# Autodesk Inventor assembly: ÜstKısım_MirrorV2
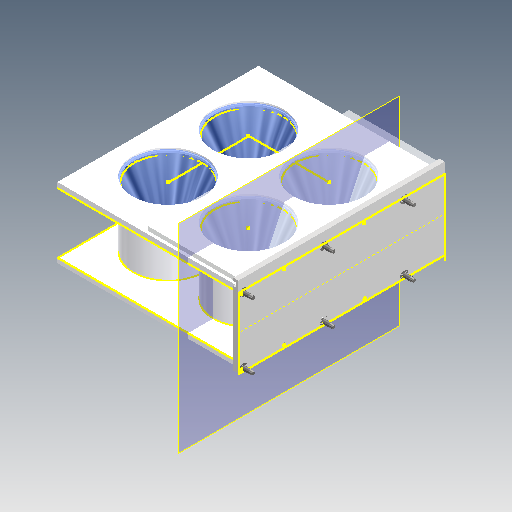
[picture p0: Inventor's stored thumbnail of the model, 512x512]
Saved by Autodesk Inventor 2020.3 (Build 243373010, 373A)
## iProperties
Created: 2020-12-03
Part Number: ÜstKısım_MirrorV2
Document SubType Name: Assembly
Designer: Yusuf
Mass: 1177.22 g
Surface Area: 3354.87 cm^2
Volume: 1142.84 cm^3
Density: 1.03007 g/cm^3
Author: Yusuf
## Documents named in this file (8)
- C:\Users\Yusuf\Desktop\SunCollector\ÜstKısım_MirrorV2.iam
- C:\Users\Yusuf\Desktop\SunCollector\Lens.ipt
- C:\Users\Yusuf\Desktop\SunCollector\LensHolder_MirrorV2.ipt
- C:\Users\Yusuf\Desktop\SunCollector\SidePanel_MirrorV2.ipt
- C:\Users\Yusuf\Documents\Inventor\Content Center Files\R2020\en-US\ANSI B18.6.5M(24)\ANSI B18.6.5M - M4x0,7 x 10(36).ipt
- C:\Users\Yusuf\Documents\Inventor\Content Center Files\R2020\en-US\ANSI B18.6.5M(23)\ANSI B18.6.5M - M6x1 x 20(39).ipt
- C:\Users\Yusuf\Desktop\SunCollector\BottomPart_MirrorV2.ipt
- C:\Users\Yusuf\Desktop\SunCollector\GlassSaver_MirrorV2.ipt
## Components (18 placed, 7 different names)
1. Lens:1 — Mate:2, Mate:1
2. LensHolder_MirrorV2:1 — Mate:2, Mate:1, Flush:2, Flush:1, Mate:10, Mate:9, Mate:8, Mate:7, Mate:4, Mate:6, Mate:5, Mate:14, Mate:13, Mate:15, Flush:3
3. SidePanel_MirrorV2:1 — Flush:2, Flush:1, Mate:10, Mate:12, Mate:11, Mate:16, Mate:18, Flush:4, Mate:17
4. Lens:2 — Mate:9, Mate:8
5. Lens:3 — Mate:7, Mate:4
6. Lens:4 — Mate:6, Mate:5
7. BottomPart_MirrorV2:1 — Mate:16, Mate:15, Flush:3
8. GlassSaver_MirrorV2:1 — Mate:18, Flush:4, Mate:17
9. Cross Recessed Pan Head Tapping Screw - Type F - Type I - Metric M4x0,7 x 10:1 — Mate:12, Mate:11
10. Cross Recessed Pan Head Tapping Screw - Type F - Type I - Metric M4x0,7 x 10:2
11. Cross Recessed Pan Head Tapping Screw - Type F - Type I - Metric M4x0,7 x 10:5
12. Cross Recessed Pan Head Tapping Screw - Type F - Type I - Metric M4x0,7 x 10:6
13. Cross Recessed Pan Head Tapping Screw - Type F - Type I - Metric M4x0,7 x 10:9
14. Cross Recessed Pan Head Tapping Screw - Type F - Type I - Metric M4x0,7 x 10:10
15. Cross Recessed Pan Head Tapping Screw - Type D - Type IA - Metric M6x1 x 20:1 — Mate:14, Mate:13
16. Cross Recessed Pan Head Tapping Screw - Type D - Type IA - Metric M6x1 x 20:2
17. Cross Recessed Pan Head Tapping Screw - Type D - Type IA - Metric M6x1 x 20:3
18. Cross Recessed Pan Head Tapping Screw - Type D - Type IA - Metric M6x1 x 20:4
## Component patterns: (10 elements, first: Cross Recessed Pan Head Tapping Screw - Type F - Type I - Metric M4x0,7 x 10:1), (4 elements, first: Cross Recessed Pan Head Tapping Screw - Type D - Type IA - Metric M6x1 x 20:1)
## Relationships (21: Mate 17, Flush 4)
- Mate:2: Lens:1 ↔ LensHolder_MirrorV2:1
- Mate:1: Lens:1 ↔ LensHolder_MirrorV2:1
- Flush:2 (-5 mm): LensHolder_MirrorV2:1 ↔ SidePanel_MirrorV2:1
- Flush:1: LensHolder_MirrorV2:1 ↔ SidePanel_MirrorV2:1
- Mate:10: LensHolder_MirrorV2:1 ↔ SidePanel_MirrorV2:1
- Mate:9: LensHolder_MirrorV2:1 ↔ Lens:2
- Mate:8: LensHolder_MirrorV2:1 ↔ Lens:2
- Mate:7: LensHolder_MirrorV2:1 ↔ Lens:3
- Mate:4: LensHolder_MirrorV2:1 ↔ Lens:3
- Mate:6: LensHolder_MirrorV2:1 ↔ Lens:4
- Mate:5: LensHolder_MirrorV2:1 ↔ Lens:4
- Mate:12: SidePanel_MirrorV2:1 ↔ Cross Recessed Pan Head Tapping Screw - Type F - Type I - Metric M4x0,7 x 10:1
- Mate:11: SidePanel_MirrorV2:1 ↔ Cross Recessed Pan Head Tapping Screw - Type F - Type I - Metric M4x0,7 x 10:1
- Mate:14: LensHolder_MirrorV2:1 ↔ Cross Recessed Pan Head Tapping Screw - Type D - Type IA - Metric M6x1 x 20:1
- Mate:13: LensHolder_MirrorV2:1 ↔ Cross Recessed Pan Head Tapping Screw - Type D - Type IA - Metric M6x1 x 20:1
- Mate:16: SidePanel_MirrorV2:1 ↔ BottomPart_MirrorV2:1
- Mate:15: LensHolder_MirrorV2:1 ↔ BottomPart_MirrorV2:1
- Flush:3: LensHolder_MirrorV2:1 ↔ BottomPart_MirrorV2:1
- Mate:18: SidePanel_MirrorV2:1 ↔ GlassSaver_MirrorV2:1
- Flush:4: SidePanel_MirrorV2:1 ↔ GlassSaver_MirrorV2:1
- Mate:17: SidePanel_MirrorV2:1 ↔ GlassSaver_MirrorV2:1
